# Autodesk Inventor assembly: MGN12H_250mm
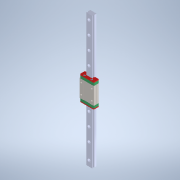
[picture p0: Inventor's stored thumbnail of the model, 180x180]
Saved by Autodesk Inventor 2020 (Build 240168000, 168)
## iProperties
Created: 2020-09-22
Part Number: MGN12H_250mm
Document SubType Name: Assembly
Designer: magnarecta
Title: C:/Users/lvglv/Downloads/MGN12H_250mm.step
Sending System: Autodesk Translation Framework v9.3.0.1241
Preprocessor: ST-DEVELOPER v18.1
## Documents named in this file (3)
- C:\Users\lvglv\Documents\GitHub\Cheap_Belt_Printer\Model\Parts\Linear_Guide\MGN12H_250mm\MGN12H_250mm.iam
- C:\Users\lvglv\Documents\GitHub\Cheap_Belt_Printer\Model\Parts\Linear_Guide\MGN12H_250mm\MGN12 LINEAR GUIDE RAIL, CONFIGURABLE, 250 mm.ipt
- C:\Users\lvglv\Documents\GitHub\Cheap_Belt_Printer\Model\Parts\Linear_Guide\MGN12H_250mm\MGN12H, LINEAR GUIDE BLOCK.ipt
## Components (2 placed, 2 different names)
1. MGN12 LINEAR GUIDE RAIL, CONFIGURABLE, 250 mm:1 — Slider:1
2. MGN12H, LINEAR GUIDE BLOCK:1 — Slider:1
## Relationships (1: TranslationJoint 1)
- Slider:1 [TranslationJoint]: MGN12 LINEAR GUIDE RAIL, CONFIGURABLE, 250 mm:1 ↔ MGN12H, LINEAR GUIDE BLOCK:1
